# Autodesk Inventor assembly: Z Axis Liner Rail Bracket Assembly - Tall - Right 1.0
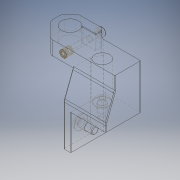
[picture p0: Inventor's stored thumbnail of the model, 180x180]
Saved by Autodesk Inventor 2016 (Build 200138000, 138)
## iProperties
Created: 2017-04-16
Part Number: Z Axis Liner Rail Bracket Assembly - Tall - Right 1.0
Document SubType Name: Assembly
Designer: Scott
Author: Scott
## Documents named in this file (5)
- E:\Scott Projects\3D Printing\CoreXY\Z Axis Liner Rail Bracket Assembly - Tall - Right 1.0.iam
- E:\Scott Projects\3D Printing\CoreXY\Z Axis Linear Rail Bracket - Double Z - Right 1.0.ipt
- E:\Scott Projects\3D Printing\CoreXY\M3 Threaded Insert.ipt
- C:\Users\Scott\Documents\Inventor\Content Center Files\R2016\en-US\ANSI B18.3.4M(1)\ANSI B18.3.4M - M5 x 0.8 x 10(2).ipt
- C:\Users\Scott\Documents\Inventor\Content Center Files\R2016\en-US\ANSI B18.3.1M(1)\ANSI B18.3.1M - M3x0.5 x 25(2).ipt
## Components (5 placed, 4 different names)
1. Z Axis Linear Rail Bracket - Double Z - Right 1.0:1 — Insert:1, Insert:2, Insert:3, Insert:4
2. M3 Threaded Insert:1 — Insert:1
3. Broached Hexagon Socket Button Head Cap Screw - Metric M5 x 0.8 x 10:1 — Insert:2
4. Broached Hexagon Socket Button Head Cap Screw - Metric M5 x 0.8 x 10:2 — Insert:3
5. Broached Socket Head Cap Screw - Metric M3x0.5 x 25:1 — Insert:4
## Relationships (4: Insert 4)
- Insert:1: Z Axis Linear Rail Bracket - Double Z - Right 1.0:1 ↔ M3 Threaded Insert:1
- Insert:2: Z Axis Linear Rail Bracket - Double Z - Right 1.0:1 ↔ Broached Hexagon Socket Button Head Cap Screw - Metric M5 x 0.8 x 10:1
- Insert:3: Z Axis Linear Rail Bracket - Double Z - Right 1.0:1 ↔ Broached Hexagon Socket Button Head Cap Screw - Metric M5 x 0.8 x 10:2
- Insert:4: Z Axis Linear Rail Bracket - Double Z - Right 1.0:1 ↔ Broached Socket Head Cap Screw - Metric M3x0.5 x 25:1
